# Autodesk Inventor assembly: wheel
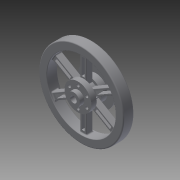
[picture p0: Inventor's stored thumbnail of the model, 180x180]
Saved by Autodesk Inventor 2014 SP1 (Build 180222100, 222)
## iProperties
Created: 2015-07-19
Part Number: wheel
Document SubType Name: Assembly
Designer: astralien3000
Author: astralien3000
## Documents named in this file (4)
- C:\Users\astralien3000\Desktop\ceres\meca\v2016\wheel.iam
- C:\Users\astralien3000\Desktop\ceres\meca\lib\wheel\pololu_wheel_80x10.ipt
- C:\Users\astralien3000\Desktop\ceres\meca\lib\struct\hub_6mm_M3.ipt
- C:\Users\astralien3000\Desktop\ceres\meca\lib\struct\poulie_rs_16T2p5s40-2.ipt
## Components (3 placed, 3 different names)
1. pololu_wheel_80x10:1 — Placage:1, Placage:2, Placage:3, Placage:4, Placage:5, Placage:6
2. hub_6mm_M3:1 — Placage:3, Placage:4
3. poulie_rs_16T2p5s40-2:1 — Placage:5, Placage:6
## Relationships (6: Mate 6)
- Placage:1 [Mate]: pololu_wheel_80x10:1
- Placage:2 [Mate]: pololu_wheel_80x10:1
- Placage:3 [Mate]: pololu_wheel_80x10:1 ↔ hub_6mm_M3:1
- Placage:4 [Mate]: pololu_wheel_80x10:1 ↔ hub_6mm_M3:1
- Placage:5 [Mate]: pololu_wheel_80x10:1 ↔ poulie_rs_16T2p5s40-2:1
- Placage:6 [Mate]: pololu_wheel_80x10:1 ↔ poulie_rs_16T2p5s40-2:1
